# Autodesk Inventor assembly: carafe_frame
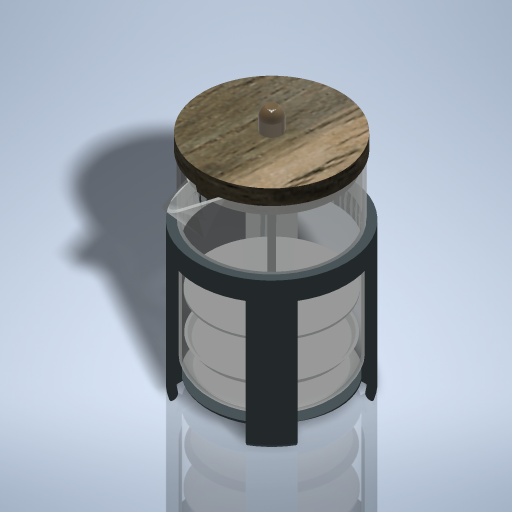
[picture p0: Inventor's stored thumbnail of the model, 512x512]
Saved by Autodesk Inventor 2024 (Build 280153000, 153)
## iProperties
Created: 2024-04-24
Part Number: carafe_frame
Document SubType Name: Assembly
Designer: ffogue
Author: ffogue
## Documents named in this file (9)
- C:\Users\ffogue\OneDrive - MuM - OM\Dokumente\Inventor\french_presser\carafe_frame.iam
- C:\Users\ffogue\OneDrive - MuM - OM\Dokumente\Inventor\french_presser\frame.ipt
- C:\Users\ffogue\OneDrive - MuM - OM\Dokumente\Inventor\french_presser\carafe.ipt
- C:\Users\ffogue\OneDrive - MuM - OM\Dokumente\Inventor\french_presser\cross_plate.ipt
- C:\Users\ffogue\OneDrive - MuM - OM\Dokumente\Inventor\french_presser\mesh filter.ipt
- C:\Users\ffogue\OneDrive - MuM - OM\Dokumente\Inventor\french_presser\rod.ipt
- C:\Users\ffogue\OneDrive - MuM - OM\Dokumente\Inventor\french_presser\spiral plate.ipt
- C:\Users\ffogue\OneDrive - MuM - OM\Dokumente\Inventor\french_presser\lid.ipt
- C:\Users\ffogue\OneDrive - MuM - OM\Dokumente\Inventor\french_presser\plunger.ipt
## Components (8 placed, 8 different names)
1. frame:1 — Einfügen:1
2. carafe:1 — Einfügen:1, Einfügen:5
3. cross_plate:1 — Einfügen:2, Einfügen:3, Einfügen:5
4. mesh filter:1 — Einfügen:2
5. rod:1 — Einfügen:3, Einfügen:4, Einfügen:6, Einfügen:7
6. spiral plate:1 — Einfügen:4
7. lid:1 — Einfügen:6
8. plunger:1 — Einfügen:7
## Relationships (7: Insert 7)
- Einfügen:1 [Insert] (-34.3 mm): frame:1 ↔ carafe:1
- Einfügen:2 [Insert] (6 mm): cross_plate:1 ↔ mesh filter:1
- Einfügen:3 [Insert] (-4 mm): cross_plate:1 ↔ rod:1
- Einfügen:4 [Insert] (-40 mm): rod:1 ↔ spiral plate:1
- Einfügen:5 [Insert] (-49 mm): carafe:1 ↔ cross_plate:1
- Einfügen:6 [Insert] (-8.45 mm): rod:1 ↔ lid:1
- Einfügen:7 [Insert] (-4 mm): rod:1 ↔ plunger:1
